# Autodesk Inventor assembly: TipMat
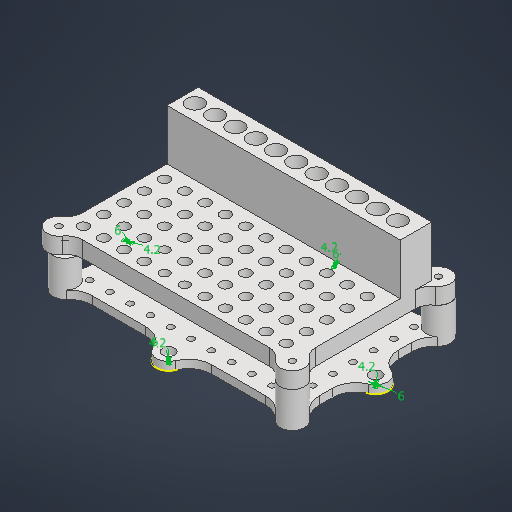
[picture p0: Inventor's stored thumbnail of the model, 512x512]
Saved by Autodesk Inventor 2025.1 (Build 291241000, 241)
## iProperties
Created: 2025-02-26
Part Number: TipMat
Document SubType Name: Assembly
Designer: m_kni
Author: m_kni
## Documents named in this file (3)
- C:\Users\jerem\Documents\GitHub\Perovskite-Automated-Synthesis-System\CAD\Tip Matrix\TipMat.iam
- C:\Users\jerem\Documents\GitHub\Perovskite-Automated-Synthesis-System\CAD\Tip Matrix\Bottom_Tip_Matrix.ipt
- C:\Users\jerem\Documents\GitHub\Perovskite-Automated-Synthesis-System\CAD\Tip Matrix\Top_Tip_Matrix.ipt
## Components (2 placed, 2 different names)
1. Bottom_Tip_Matrix:1 — Insert:1
2. Top_Tip_Matrix:1 — Insert:1
## Relationships (1: Insert 1)
- Insert:1: Bottom_Tip_Matrix:1 ↔ Top_Tip_Matrix:1
